# Autodesk Inventor assembly: Ensamblaje_Carrito
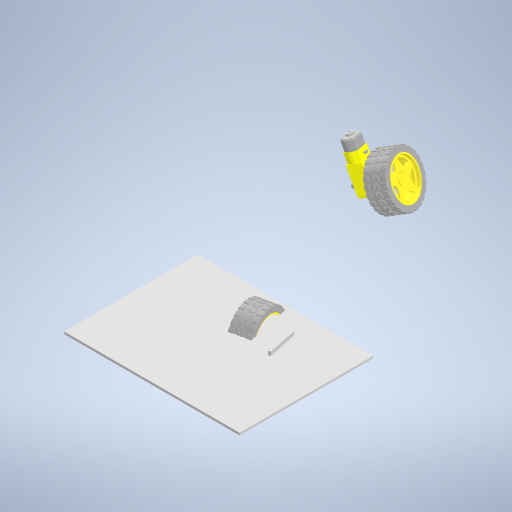
[picture p0: Inventor's stored thumbnail of the model, 512x512]
Saved by Autodesk Inventor 2024 (Build 280153000, 153)
## iProperties
Created: 2025-05-13
Part Number: Ensamblaje_Carrito
Document SubType Name: Assembly
Designer: mario
Author: mario
## Documents named in this file (4)
- C:\Programacion-de-Microcontroladores\Proyecto2\RepositorioProyecto2\Proyecto2_ModelosCAD\Ensamblaje_Carrito.iam
- C:\Programacion-de-Microcontroladores\Proyecto2\RepositorioProyecto2\Proyecto2_ModelosCAD\Importados\Ensamble de llanta v1\Ensamble de llanta v1.iam
- C:\Users\mario\OneDrive - UVG\Documentos\QUETZAL-2\Base_Carro.ipt
- C:\Users\mario\OneDrive - UVG\Documentos\QUETZAL-2\Soporte_Motorreductor.ipt
## Components (4 placed, 3 different names)
1. Ensamble de llanta v1:1 [sub-assembly] — Coincidencia:1, Coincidencia:2, Coincidencia:4
2. Ensamble de llanta v1:2 [sub-assembly]
3. Base_Carro:1 — Coincidencia:1, Coincidencia:3
4. Soporte_Motorreductor:1 — Coincidencia:2, Coincidencia:3, Coincidencia:4
## Relationships (4: Mate 4)
- Coincidencia:1 [Mate]: Ensamble de llanta v1:1 ↔ Base_Carro:1
- Coincidencia:2 [Mate]: Ensamble de llanta v1:1 ↔ Soporte_Motorreductor:1
- Coincidencia:3 [Mate]: Base_Carro:1 ↔ Soporte_Motorreductor:1
- Coincidencia:4 [Mate]: Ensamble de llanta v1:1 ↔ Soporte_Motorreductor:1
